# Autodesk Inventor assembly: Drive in a Day Frame 2013 tube example
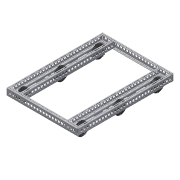
[picture p0: Inventor's stored thumbnail of the model, 180x180]
Saved by Autodesk Inventor 2013 (Build 170138000, 138)
## iProperties
Created: 2013-05-20
Part Number: Drive in a Day Frame 2013 tube example
Document SubType Name: Assembly
Designer: Nemo
Mass: 3130.52 g
Surface Area: 8744.38 cm^2
Volume: 1155.18 cm^3
Density: 2.71 g/cm^3
Author: Nemo
## Documents named in this file (5)
- H:\Nemo\Documents\Robotics\COTS Parts\Drive in a Day\Drive in a Day Frame 2013 tube example.iam
- H:\Nemo\Documents\Robotics\COTS Parts\Drive in a Day\217-2593-002 Rev3 Front-Back.ipt
- H:\Nemo\Documents\Robotics\COTS Parts\Drive in a Day\217-2593-001 Rev3 Side Rail.ipt
- H:\Nemo\Documents\Robotics\COTS Parts\Drive in a Day\VersaWheel 2 sprockets for Drive in a Day 2013.iam
- H:\Nemo\Documents\Robotics\COTS Parts\Drive in a Day\VersaWheel 2 sprockets center wheel for Drive in a Day 2013.iam
## Components (12 placed, 8 different names)
1. 217-2593-002 Rev3 Front — Flush:1, Mate:1, Mate:2, Flush:2, Insert:1, Flush:5
2. 217-2593-002 Rev3 Back — Flush:1, Mate:1, Mate:3, Mate:4
3. 217-2593-001 Rev3 Left outside — Mate:2, Flush:2, Mate:3, Mate:8, Flush:4, Flush:6, Mate:9, Mate:10, Insert:3, Insert:4
4. 217-2593-001 Rev3 Left inside — Mate:8, Flush:4, Mate:10
5. 217-2593-001 Rev3 Right outside — Insert:1, Mate:4, Flush:3, Mate:7, Mate:11, Insert:5, Insert:6, Insert:7
6. 217-2593-001 Rev3 Right inside — Flush:3, Mate:7, Mate:11
7. VersaWheel 2 sprockets for Drive in a Day 2013:2 [sub-assembly] — Insert:4, Flush:10
8. VersaWheel 2 sprockets for Drive in a Day 2013:3 [sub-assembly] — Insert:3
9. VersaWheel 2 sprockets for Drive in a Day 2013:4 [sub-assembly] — Insert:6
10. VersaWheel 2 sprockets for Drive in a Day 2013:5 [sub-assembly] — Insert:7
11. VersaWheel 2 sprockets for Drive in a Day 2013:6 [sub-assembly] — Insert:5
12. VersaWheel 2 sprockets center wheel for Drive in a Day 2013:1 [sub-assembly] — Flush:10
## Relationships (22: Mate 9, Flush 7, Insert 6)
- Flush:1: 217-2593-002 Rev3 Front ↔ 217-2593-002 Rev3 Back
- Mate:1: 217-2593-002 Rev3 Front ↔ 217-2593-002 Rev3 Back
- Mate:2: 217-2593-002 Rev3 Front ↔ 217-2593-001 Rev3 Left outside
- Flush:2: 217-2593-002 Rev3 Front ↔ 217-2593-001 Rev3 Left outside
- Mate:3: 217-2593-002 Rev3 Back ↔ 217-2593-001 Rev3 Left outside
- Insert:1: 217-2593-002 Rev3 Front ↔ 217-2593-001 Rev3 Right outside
- Mate:4: 217-2593-002 Rev3 Back ↔ 217-2593-001 Rev3 Right outside
- Flush:3: 217-2593-001 Rev3 Right outside ↔ 217-2593-001 Rev3 Right inside
- Mate:7: 217-2593-001 Rev3 Right outside ↔ 217-2593-001 Rev3 Right inside
- Mate:8: 217-2593-001 Rev3 Left outside ↔ 217-2593-001 Rev3 Left inside
- Flush:4: 217-2593-001 Rev3 Left outside ↔ 217-2593-001 Rev3 Left inside
- Flush:5: 217-2593-002 Rev3 Front
- Flush:6: 217-2593-001 Rev3 Left outside
- Mate:9 (43.815 mm): 217-2593-001 Rev3 Left outside
- Mate:10 (63.5 mm): 217-2593-001 Rev3 Left outside ↔ 217-2593-001 Rev3 Left inside
- Mate:11 (63.5 mm): 217-2593-001 Rev3 Right outside ↔ 217-2593-001 Rev3 Right inside
- Insert:3: 217-2593-001 Rev3 Left outside ↔ VersaWheel 2 sprockets for Drive in a Day 2013:3
- Insert:4: 217-2593-001 Rev3 Left outside ↔ VersaWheel 2 sprockets for Drive in a Day 2013:2
- Insert:5: 217-2593-001 Rev3 Right outside ↔ VersaWheel 2 sprockets for Drive in a Day 2013:6
- Insert:6: 217-2593-001 Rev3 Right outside ↔ VersaWheel 2 sprockets for Drive in a Day 2013:4
- Insert:7: 217-2593-001 Rev3 Right outside ↔ VersaWheel 2 sprockets for Drive in a Day 2013:5
- Flush:10: VersaWheel 2 sprockets for Drive in a Day 2013:2 ↔ VersaWheel 2 sprockets center wheel for Drive in a Day 2013:1
